# Autodesk Inventor assembly: pot__assembly_test_v1
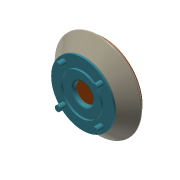
[picture p0: Inventor's stored thumbnail of the model, 180x180]
Saved by Autodesk Inventor 2017 (Build 210142000, 142)
## iProperties
Created: 2018-10-30
Part Number: pot__assembly_test_v1
Document SubType Name: Assembly
Designer: mfans
Author: mfans
## Documents named in this file (4)
- C:\Users\mfans\Dropbox (Startup Shell)\codeProjects\holonomic-plant-pot\cad\mounting\pot\pot__assembly_test_v1.iam
- C:\Users\mfans\Dropbox (Startup Shell)\codeProjects\holonomic-plant-pot\cad\mounting\pot\sensor_holder.ipt
- C:\Users\mfans\Dropbox (Startup Shell)\codeProjects\holonomic-plant-pot\cad\mounting\pot\pot_holder_prototype.ipt
- C:\Users\mfans\Dropbox (Startup Shell)\codeProjects\holonomic-plant-pot\cad\mounting\pot\pot_base_adapter2.ipt
## Components (3 placed, 3 different names)
1. sensor_holder:1 — Insert:1, Mate:1, Mate:2, Mate:3
2. pot_holder_prototype:1 — Insert:1
3. pot_base_adapter2:1 — Mate:1, Mate:2, Mate:3
## Relationships (4: Mate 3, Insert 1)
- Insert:1 (8.5 mm): sensor_holder:1 ↔ pot_holder_prototype:1
- Mate:1 (0.25 mm): sensor_holder:1 ↔ pot_base_adapter2:1
- Mate:2 (0.25 mm): sensor_holder:1 ↔ pot_base_adapter2:1
- Mate:3: sensor_holder:1 ↔ pot_base_adapter2:1
